# Autodesk Inventor assembly: ASY TZS 1752 FDS way 2
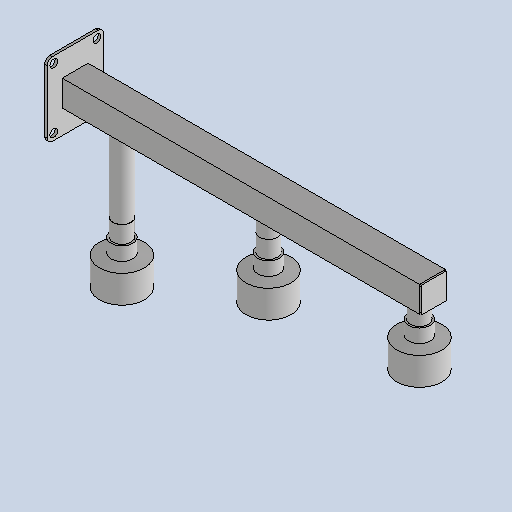
[picture p0: Inventor's stored thumbnail of the model, 512x512]
Saved by Autodesk Inventor 2025.1 (Build 291241020, 241B)
## iProperties
Created: 2025-07-02
Part Number: ASY TZS 1752 FDS way 2
Document SubType Name: Assembly
Designer: user
Author: user
## Documents named in this file (8)
- C:\Users\pokla\Documents\Inventor\TZS-Tazovskiy\Filter D1200\FDS\ASY TZS 1752 FDS way 2.iam
- C:\Users\pokla\Documents\Inventor\TZS-Tazovskiy\Filter D1200\FDS\TZS 1752 FDS 1200 way tube 2.ipt
- C:\Users\pokla\Documents\Inventor\TZS-Tazovskiy\Filter D1200\FDS\TZS dummy filter element.ipt
- C:\Users\pokla\Documents\Inventor\TZS-Tazovskiy\Filter D1200\FDS\TZS dummy pipe nippel.ipt
- C:\Users\pokla\Documents\Inventor\TZS-Tazovskiy\Filter D1200\FDS\TZS 1756 FDS 1200 way tube 6.ipt
- C:\Users\pokla\Documents\Inventor\TZS-Tazovskiy\Filter D1200\FDS\TZS 1757 FDS 1200 way tube 7.ipt
- C:\Users\pokla\Documents\Inventor\TZS-Tazovskiy\Filter D1200\FDS\TZS 760 FDS 1200 FLANGE 3.ipt
- C:\Users\pokla\Documents\Inventor\TZS-Tazovskiy\Filter D1200\FDS\TZS 766 FDS 1200 CUP 1.ipt
## Components (11 placed, 7 different names)
1. PNS 755 FDS 1200 way tube 2.ipt:1
2. PNS dummy filter element.ipt:1
3. PNS dummy pipe nippel.ipt:1
4. PNS 758 FDS 1200 way tube 6.ipt:1
5. PNS dummy filter element.ipt:2
6. PNS dummy pipe nippel.ipt:2
7. PNS 759 FDS 1200 way tube 7.ipt:1
8. PNS dummy filter element.ipt:3
9. PNS dummy pipe nippel.ipt:3
10. PNS 760 FDS 1200 FLANGE 3.ipt:1
11. PNS 766 FDS 1200 CUP 1.ipt:1
## Relationships (10: WeldJoint 10)
- [WeldJoint]: PNS dummy filter element.ipt:1 ↔ PNS dummy pipe nippel.ipt:1
- [WeldJoint]: PNS 755 FDS 1200 way tube 2.ipt:1 ↔ PNS dummy pipe nippel.ipt:1
- [WeldJoint]: PNS dummy filter element.ipt:2 ↔ PNS dummy pipe nippel.ipt:2
- [WeldJoint]: PNS 758 FDS 1200 way tube 6.ipt:1 ↔ PNS dummy pipe nippel.ipt:2
- [WeldJoint]: PNS 755 FDS 1200 way tube 2.ipt:1 ↔ PNS 758 FDS 1200 way tube 6.ipt:1
- [WeldJoint]: PNS dummy filter element.ipt:3 ↔ PNS dummy pipe nippel.ipt:3
- [WeldJoint]: PNS 759 FDS 1200 way tube 7.ipt:1 ↔ PNS dummy pipe nippel.ipt:3
- [WeldJoint]: PNS 755 FDS 1200 way tube 2.ipt:1 ↔ PNS 759 FDS 1200 way tube 7.ipt:1
- [WeldJoint] (-3 mm): PNS 755 FDS 1200 way tube 2.ipt:1 ↔ PNS 760 FDS 1200 FLANGE 3.ipt:1
- [WeldJoint]: PNS 755 FDS 1200 way tube 2.ipt:1 ↔ PNS 766 FDS 1200 CUP 1.ipt:1
## Named parameters: d40_d37_d34_d31 = 0 mm, d49_d45_d43_d40_d37_d34_d31 = 0 mm, d50_d46 = 0 mm
